# Autodesk Inventor assembly: GearBox and Grip
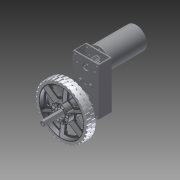
[picture p0: Inventor's stored thumbnail of the model, 180x180]
Saved by Autodesk Inventor 2015 (Build 190159000, 159)
## iProperties
Created: 2016-01-10
Part Number: GearBox and Grip
Document SubType Name: Assembly
Designer: Applefamily
Author: Applefamily
## Documents named in this file (3)
- C:\Users\Applegate\Desktop\Chassy_Wheeled\Assembly\GearBox and Grip.iam
- C:\Users\Applegate\Desktop\Chassy_Wheeled\Assembly\Imported Components\Toughbox+Nano+All+Shafts+v2\Toughbox+Nano+All+Shafts+v2.iam
- C:\Users\Applegate\Downloads\Imported Components\am-940a-6-HiGrip-\am-940a-6-HiGrip-.iam
## Components (2 placed, 2 different names)
1. Toughbox+Nano+All+Shafts+v2:1 [sub-assembly] — Cylindrical:1
2. am-940a-6-HiGrip-:1 [sub-assembly] — Cylindrical:1
## Relationships (1: CylindricalJoint 1)
- Cylindrical:1: Toughbox+Nano+All+Shafts+v2:1 ↔ am-940a-6-HiGrip-:1
